# Autodesk Inventor assembly: 123
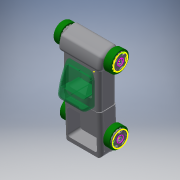
[picture p0: Inventor's stored thumbnail of the model, 180x180]
Saved by Autodesk Inventor 2018 (Build 220112000, 112)
## iProperties
Created: 2019-04-04
Part Number: 123
Document SubType Name: Assembly
Designer: This kid
Author: This kid
## Documents named in this file (9)
- D:\Users\russd\Documents\GitHub\IED-files\123.iam
- D:\Users\russd\Documents\GitHub\IED-files\5.5\5.5a\ARTHURW5.5a AXLE.ipt
- D:\Users\russd\Documents\GitHub\IED-files\5.5\5.5a\AWAutomobloxTire.ipt
- D:\Users\russd\Documents\GitHub\IED-files\5.5\5.5b\ARTHURw5.5bAutomobloxConnectorPiece.ipt
- D:\Users\russd\Documents\GitHub\IED-files\5.2\5.2b\AW5.2bWINDSHIELD.ipt
- D:\Users\russd\Documents\GitHub\IED-files\5.2\5.2b\AutomobloxWheel.ipt
- D:\T9 Passenger Section (1).ipt
- D:\Users\russd\Documents\GitHub\IED-files\Autoblox front.ipt
- D:\T9 Bed.ipt
## Components (17 placed, 8 different names)
1. AWAutomobloxTire:1 — Mate:2
2. ARTHURw5.5bAutomobloxConnectorPiece:1 — Mate:11
3. AW5.2bWINDSHIELD:1 — Mate:13
4. AutomobloxWheel:1 — Mate:2
5. AWAutomobloxTire:2
6. AutomobloxWheel:2
7. AWAutomobloxTire:3
8. AutomobloxWheel:3
9. ARTHURW5.5a AXLE:4
10. AWAutomobloxTire:4 — Mate:21
11. AutomobloxWheel:4 — Mate:21
12. AWAutomobloxTire:5
13. AutomobloxWheel:5
14. T9 Passenger Section (1):1 — Mate:11, Mate:13, Mate:14, Mate:19
15. ARTHURw5.5bAutomobloxConnectorPiece:2 — Mate:14, Mate:17, Mate:18
16. Autoblox front:1 — Mate:17, Mate:18
17. T9 Bed:1 — Mate:19
## Relationships (13: Mate 13)
- Mate:2: AWAutomobloxTire:1 ↔ AutomobloxWheel:1
- [Mate]: AWAutomobloxTire:2 ↔ AutomobloxWheel:2
- [Mate]: AWAutomobloxTire:3 ↔ AutomobloxWheel:3
- [Mate]: ARTHURW5.5a AXLE:4 ↔ AutomobloxWheel:4
- [Mate]: AWAutomobloxTire:4 ↔ AutomobloxWheel:4
- [Mate]: AWAutomobloxTire:5 ↔ AutomobloxWheel:5
- Mate:11: ARTHURw5.5bAutomobloxConnectorPiece:1 ↔ T9 Passenger Section (1):1
- Mate:13: AW5.2bWINDSHIELD:1 ↔ T9 Passenger Section (1):1
- Mate:14: T9 Passenger Section (1):1 ↔ ARTHURw5.5bAutomobloxConnectorPiece:2
- Mate:17: ARTHURw5.5bAutomobloxConnectorPiece:2 ↔ Autoblox front:1
- Mate:18: ARTHURw5.5bAutomobloxConnectorPiece:2 ↔ Autoblox front:1
- Mate:19: T9 Passenger Section (1):1 ↔ T9 Bed:1
- Mate:21: AWAutomobloxTire:4 ↔ AutomobloxWheel:4
## Named parameters: d3_d1 = 0 mm, d5_d1 = 0 mm, d6_d0 = 0 mm, d7_d1 = 0 mm, d9_d1 = 0 mm
